# Autodesk Inventor assembly: prototype1
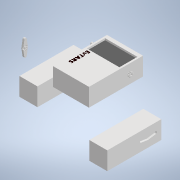
[picture p0: Inventor's stored thumbnail of the model, 180x180]
Saved by Autodesk Inventor 2021 (Build 250183000, 183)
## iProperties
Created: 2025-04-02
Part Number: prototype1
Document SubType Name: Assembly
Designer: Admin
Author: Admin
## Documents named in this file (4)
- C:\Users\Admin\Documents\file inventor 3d\robot TARS\prototype1.iam
- C:\Users\Admin\Documents\file inventor 3d\robot TARS\body.ipt
- C:\Users\Admin\Documents\file inventor 3d\robot TARS\tangan kanan.ipt
- C:\Users\Admin\Documents\file inventor 3d\robot TARS\servo horn.ipt
## Components (5 placed, 4 different names)
1. body:1 — Mate:1
2. tangan kiri:1
3. tangan kanan:2
4. servo horn:1
5. servo horn:2 — Mate:1
## Relationships (1: Mate 1)
- Mate:1: body:1 ↔ servo horn:2
